# Autodesk Inventor assembly: Arrm
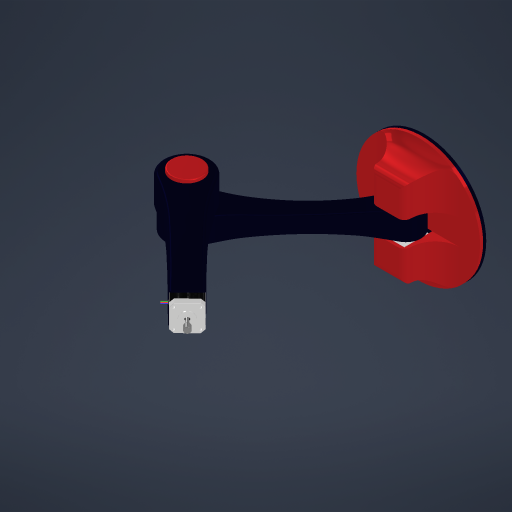
[picture p0: Inventor's stored thumbnail of the model, 512x512]
Saved by Autodesk Inventor 2023 (Build 270158000, 158)
## iProperties
Created: 2023-04-09
Part Number: Arrm
Document SubType Name: Assembly
Designer: vatdu
Author: vatdu
## Documents named in this file (3)
- C:\Users\vatdu\Desktop\CRYSTAL MARK II\Arm\Arrm.iam
- C:\Users\vatdu\Desktop\CRYSTAL MARK II\Arm\Shoulder\Shoulder V2.iam
- C:\Users\vatdu\Desktop\CRYSTAL MARK II\Arm\Elbow\Elbow.iam
## Components (2 placed, 2 different names)
1. Shoulder V2:1 [sub-assembly] — Rotational:1
2. Elbow:1 [sub-assembly] — Rotational:1
## Relationships (1: RevoluteJoint 1)
- Rotational:1 [RevoluteJoint]: Shoulder V2:1 ↔ Elbow:1
